# Autodesk Inventor assembly: sg90 long claw
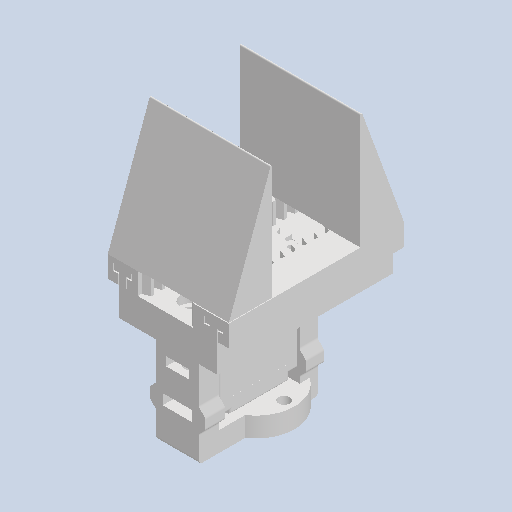
[picture p0: Inventor's stored thumbnail of the model, 512x512]
Saved by Autodesk Inventor 2025 (Build 290162000, 162)
## iProperties
Created: 2025-06-09
Part Number: sg90 long claw
Document SubType Name: Assembly
Designer: gavin
Author: gavin
## Documents named in this file (6)
- D:\Inventor\robot armT 2\sg90 long claw.iam
- D:\Inventor\robot armT 2\9G Servo Motor SG90.ipt
- D:\Inventor\robot armT 2\sg90 claw v2.ipt
- D:\Inventor\robot armT 2\sg90 claw v2 gear m1.ipt
- D:\Inventor\robot armT 2\sg90 claw v2 holder.ipt
- D:\Inventor\robot armT 2\sg90 claw finger long.ipt
## Components (6 placed, 5 different names)
1. 9G Servo Motor SG90:1 — 貼合:8, 貼合:9, 貼合:10
2. sg90 claw v2:1 — 貼合:10, 齊平:3, 齊平:4
3. sg90 claw v2 gear m1:1
4. sg90 claw v2 holder:1 — 貼合:8, 貼合:9
5. sg90 claw finger long:1 — 齊平:3
6. sg90 claw finger long:2 — 齊平:4
## Relationships (14: Mate 10, Flush 4)
- [Flush]: 9G Servo Motor SG90:1 ↔ sg90 claw v2:1
- [Mate]: 9G Servo Motor SG90:1 ↔ sg90 claw v2 gear m1:1
- [Mate]: 9G Servo Motor SG90:1 ↔ sg90 claw v2 gear m1:1
- [Mate]: 9G Servo Motor SG90:1 ↔ sg90 claw v2:1
- [Flush]: 9G Servo Motor SG90:1 ↔ sg90 claw v2 holder:1
- [Mate]: sg90 claw v2:1 ↔ sg90 claw finger long:1
- [Mate] (0.2 mm): sg90 claw v2:1 ↔ sg90 claw finger long:1
- [Mate]: sg90 claw v2:1 ↔ sg90 claw finger long:2
- [Mate] (0.2 mm): sg90 claw v2:1 ↔ sg90 claw finger long:2
- 貼合:8 [Mate]: 9G Servo Motor SG90:1 ↔ sg90 claw v2 holder:1
- 貼合:9 [Mate]: 9G Servo Motor SG90:1 ↔ sg90 claw v2 holder:1
- 貼合:10 [Mate]: 9G Servo Motor SG90:1 ↔ sg90 claw v2:1
- 齊平:3 [Flush]: sg90 claw v2:1 ↔ sg90 claw finger long:1
- 齊平:4 [Flush]: sg90 claw v2:1 ↔ sg90 claw finger long:2
